# Autodesk Inventor assembly: SG90 - Micro Servo 9g - Tower Pro
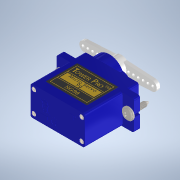
[picture p0: Inventor's stored thumbnail of the model, 180x180]
Saved by Autodesk Inventor 2020.1 (Build 241239000, 239)
## iProperties
Created: 2017-11-11
Part Number: SG90 - Micro Servo 9g - Tower Pro
Document SubType Name: Assembly
Designer: Daniel
Sending System: SolidWorks 2016
Last Author: mathe
Last Saved: 2017-11-11
Peso: 10.17
Projetista: Matheus A. Frasson
Data do Projeto: 00/00/0000
Data de Aprovação: 00/00/0000
Quantidade: 01
Revisão: Matheus A. Frasson
Aprovação: Matheus A. Frasson
Custo Total: 0.00
Author: Daniel
## Documents named in this file (5)
- F:\Proyectos\Dog Feeder\Solido\Servo SG90\SG90 - Micro Servo 9g - Tower Pro.iam
- F:\Proyectos\Dog Feeder\Solido\Servo SG90\SG90 - Micro Servo 9g - Tower Pro.1.ipt
- F:\Proyectos\Dog Feeder\Solido\Servo SG90\SG90 - Micro Servo 9g - Tower Pro.3.ipt
- F:\Proyectos\Dog Feeder\Solido\Servo SG90\SG90 - Micro Servo 9g - Tower Pro.5.ipt
- F:\Proyectos\Dog Feeder\Solido\Servo SG90\SG90 - Micro Servo 9g - Tower Pro.6.ipt
## Components (5 placed, 4 different names)
1. Tower Pro - Micro Servo 9g - SG90.1:1 — Mate:1, Mate:2
2. SG90 - Micro Servo 9g - Tower Pro.3:1
3. SG90 - Micro Servo 9g - Tower Pro.5:1 — Mate:1
4. SG90 - Micro Servo 9g - Tower Pro.5:2 — Mate:2
5. SG90 - Micro Servo 9g - Tower Pro.6:1
## Relationships (2: Mate 2)
- Mate:1: Tower Pro - Micro Servo 9g - SG90.1:1 ↔ SG90 - Micro Servo 9g - Tower Pro.5:1
- Mate:2: Tower Pro - Micro Servo 9g - SG90.1:1 ↔ SG90 - Micro Servo 9g - Tower Pro.5:2
